# Autodesk Inventor assembly: HutesHocsereloEsBorda
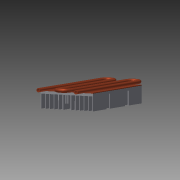
[picture p0: Inventor's stored thumbnail of the model, 180x180]
Saved by Autodesk Inventor 2015 (Build 190159000, 159)
## iProperties
Created: 2014-11-06
Part Number: HutesHocsereloEsBorda
Document SubType Name: Assembly
Designer: laca
Author: laca
## Documents named in this file (3)
- C:\Users\laca\Documents\inventor\iRoobo2014Ver3\HutesHocsereloEsBorda.iam
- C:\Users\laca\Documents\inventor\iRoobo2014Ver3\HutoBorda.ipt
- C:\Users\laca\Documents\inventor\iRoobo2014Ver3\RezLemezHocserelo.ipt
## Components (2 placed, 2 different names)
1. HutoBorda:1 — Rotational:1, Rotational:2
2. RezLemezHocserelo:1 — Rotational:1, Rotational:2
## Relationships (2: RevoluteJoint 2)
- Rotational:1 [RevoluteJoint]: HutoBorda:1 ↔ RezLemezHocserelo:1
- Rotational:2 [RevoluteJoint]: HutoBorda:1 ↔ RezLemezHocserelo:1
